# Autodesk Inventor assembly: 1054.000(2)
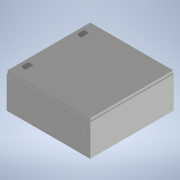
[picture p0: Inventor's stored thumbnail of the model, 180x180]
Saved by Autodesk Inventor 2021 (Build 250183000, 183)
## iProperties
Category: PARTsolutions
Company: RITTAL
Created: 2025-08-26
Part Number: 1054.000(2)
Catalog Web Link: www.cadenas.de
Description: AX Compact enclosure-sheet steel
Vendor: RITTAL
Document SubType Name: Assembly
Designer: psAdmin
Manufacturer: RITTAL
Mass: 3196.97 g
Surface Area: 36267.6 cm^2
Volume: 3196.97 cm^3
Density: 1 g/cm^3
Title: 1054.000(2)
Author: Cadenas PARTsolutions
Comments: sheet steel
PSOL_IDENT_0: {$CADENAS_DATA/23d-libs/rittal/schaltschranksys/kompakt_schaltschr/ae_2_0_asmtab.prj},203 {VTYP=3D},
PSOL_IDENT_1: {STYP=ASSTAB},{NB=1054.000(2)},{LINA=1054.000(2)},{NN=AX Compact enclosure},{DATE=28.04.2025 21:11:2
PSOL_IDENT_2: 3},{GEOMDATE=11.04.2025 11:21:44},{VERSION=},{LINEID=340},{WBVAR=DETAIL},{WBNUMERIC=DETAIL}  {NB=105
PSOL_IDENT_3: 4.000(2)},{LINA=1054.000(2)},{KT=DUMMY},{BEST=1054.000},{BEM=2},{DETAIL=2},{INFOWWW=Website},{BEZ1=A
PSOL_IDENT_4: X Kompakt-Schaltschrank},{BEZ2=Stahlblech},{BEZ3=eintürig},{INFO=Überarbeitete Version 11/2024},{B=6
PSOL_IDENT_5: 00},{H=600},{T=250},{F=550},{G=575},{B1=600},{H1=600},{T1=250},{F1=550},{G1=575},{S=2.5},{ST=MIN},{G
PSOL_IDENT_6: EW=23,4},{VERS=34},{CNSECLASS51=27-18-01-02},{CNSECLASS70=27-18-01-01},{CNSECLASS80=27-18-01-01},{CN
PSOL_IDENT_7: SETIM40=EC000261},{PPATH=assemblies_ae_2_0/ae_2_0_asmtpl.prj},{INFOPAGE=ax_s30},{INFOPATH=http://www
PSOL_IDENT_8: .rittal.com/de-de/part/1054000},{BESTE1=1054},{BESTE2=000},{DETAIL1= 2, 'niedrig', 'detail_2.png', 1
PSOL_IDENT_9: , 'hoch', 'detail_1.png', 11  , 'hochsperr', 'detail_11.png'},{CNSETIM80=EC000261},{CNSETIM90=EC0002
PSOL_IDENT_10: 61},{CNSECLASS60=27-18-01-01},{UNSPSC=31-26-15-02}
NB: 1054.000(2)
NN: AX Compact enclosure
NT: sheet steel
NBSYN: $BEST.($DETAIL.)
LINA: 1054.000(2)
CATALOG: Rittal
BEST: 1054.000
DETAIL: low
INFOWWW: webseite
BEZ1: AX Compact enclosure
BEZ2: sheet steel
BEZ3: single door
INFO: Revised version 11/2024
B: 600
H: 600
T: 250
F: 550
G: 575
GEW: 23,4
CNSECLASS70: 27-18-01-01
CNSECLASS80: 27-18-01-01
CNSETIM80: EC000261
CNSETIM90: EC000261
CNSECLASS60: 27-18-01-01
UNSPSC: 31-26-15-02
SUPPLIER: RITTAL
ARTICLENO: 1054.000(2)
BOMINFO: 1054.000(2)
CREATOR: CADENAS GmbH
## Documents named in this file (9)
- e:\temp\worker_COMMON_247\temp\tmp_5808_86_FYTeN\format_0\1054_000(2).iam
- e:\temp\worker_COMMON_247\temp\tmp_5808_86_FYTeN\format_0\1054_000(2)_P1.ipt
- e:\temp\worker_COMMON_247\temp\tmp_5808_86_FYTeN\format_0\1XXX_01_04(B,2)_P7.ipt
- e:\temp\worker_COMMON_247\temp\tmp_5808_86_FYTeN\format_0\1XXX_01_04(T,2)_P7.ipt
- e:\temp\worker_COMMON_247\temp\tmp_5808_86_FYTeN\format_0\166X_01_01(2)_P2.ipt
- e:\temp\worker_COMMON_247\temp\tmp_5808_86_FYTeN\format_0\1XXX_01_05(2)_P8.ipt
- e:\temp\worker_COMMON_247\temp\tmp_5808_86_FYTeN\format_0\1XX7_04_00_7(2)_P5.ipt
- e:\temp\worker_COMMON_247\temp\tmp_5808_86_FYTeN\format_0\166X_02_00_P6_(2).ipt
- e:\temp\worker_COMMON_247\temp\tmp_5808_86_FYTeN\format_0\0000-00168553(2).ipt
## Components (9 placed, 8 different names)
1. 1054_000(2)_P1:1 — SCRO_XY@1 <-> SC_XY@2, SCRO_Z@1 <-> SC_Z@2, SCRO_YZ@1 <-> SC_YZ@2, SCRU_XY@1 <-> SC_XY@3, SCRU_Z@1 <-> SC_Z@3, SCRU_YZ@1 <-> SC_YZ@3, FP1_XY@1 <-> FP_XY@7, FP1_Z@1 <-> FP_Z@7, FP1_YZ@1 <-> FP_YZ@7, MP_XY@1 <-> MP_XY@8, MP_Z@1 <-> MP_Z@8, MP_YZ@1 <-> MP_YZ@8, to_Plug_XY@1 <-> P1_XY@9, to_Plug_Z@1 <-> P1_Z@9, to_Plug_YZ@1 <-> P1_YZ@9
2. 1XXX_01_04(B,2)_P7:1 — SCRO_XY@1 <-> SC_XY@2, SCRO_Z@1 <-> SC_Z@2, SCRO_YZ@1 <-> SC_YZ@2
3. 1XXX_01_04(T,2)_P7:1 — SCRU_XY@1 <-> SC_XY@3, SCRU_Z@1 <-> SC_Z@3, SCRU_YZ@1 <-> SC_YZ@3, TUER2_XY@3 <-> ET_XY@4, TUER2_Z@3 <-> ET_Z@4
4. 166X_01_01(2)_P2:1 — TUER2_XY@3 <-> ET_XY@4, TUER2_Z@3 <-> ET_Z@4, VV1_XY@4 <-> VV_XY@5, VV1_Z@4 <-> VV_Z@5, VV1_YZ@4 <-> VV_YZ@5, VV2_XY@4 <-> VV_XY@6, VV2_Z@4 <-> VV_Z@6, VV2_YZ@4 <-> VV_YZ@6
5. 1XXX_01_05(2)_P8:1 — VV1_XY@4 <-> VV_XY@5, VV1_Z@4 <-> VV_Z@5, VV1_YZ@4 <-> VV_YZ@5
6. 1XXX_01_05(2)_P8:2 — VV2_XY@4 <-> VV_XY@6, VV2_Z@4 <-> VV_Z@6, VV2_YZ@4 <-> VV_YZ@6
7. 1XX7_04_00_7(2)_P5:1 — FP1_XY@1 <-> FP_XY@7, FP1_Z@1 <-> FP_Z@7, FP1_YZ@1 <-> FP_YZ@7
8. 166X_02_00_P6_(2):1 — MP_XY@1 <-> MP_XY@8, MP_Z@1 <-> MP_Z@8, MP_YZ@1 <-> MP_YZ@8
9. 0000-00168553(2):1 — to_Plug_XY@1 <-> P1_XY@9, to_Plug_Z@1 <-> P1_Z@9, to_Plug_YZ@1 <-> P1_YZ@9
## Relationships (23: Mate 15, Angle 7, Flush 1)
- SCRO_XY@1 <-> SC_XY@2 [Mate]: 1054_000(2)_P1:1 ↔ 1XXX_01_04(B,2)_P7:1
- SCRO_Z@1 <-> SC_Z@2 [Mate]: 1054_000(2)_P1:1 ↔ 1XXX_01_04(B,2)_P7:1
- SCRO_YZ@1 <-> SC_YZ@2 [Angle] (0 deg): 1054_000(2)_P1:1 ↔ 1XXX_01_04(B,2)_P7:1
- SCRU_XY@1 <-> SC_XY@3 [Mate]: 1054_000(2)_P1:1 ↔ 1XXX_01_04(T,2)_P7:1
- SCRU_Z@1 <-> SC_Z@3 [Mate]: 1054_000(2)_P1:1 ↔ 1XXX_01_04(T,2)_P7:1
- SCRU_YZ@1 <-> SC_YZ@3 [Angle] (0 deg): 1054_000(2)_P1:1 ↔ 1XXX_01_04(T,2)_P7:1
- TUER2_XY@3 <-> ET_XY@4 [Mate]: 1XXX_01_04(T,2)_P7:1 ↔ 166X_01_01(2)_P2:1
- TUER2_Z@3 <-> ET_Z@4 [Mate]: 1XXX_01_04(T,2)_P7:1 ↔ 166X_01_01(2)_P2:1
- VV1_XY@4 <-> VV_XY@5 [Mate]: 166X_01_01(2)_P2:1 ↔ 1XXX_01_05(2)_P8:1
- VV1_Z@4 <-> VV_Z@5 [Mate]: 166X_01_01(2)_P2:1 ↔ 1XXX_01_05(2)_P8:1
- VV1_YZ@4 <-> VV_YZ@5 [Angle] (0 deg): 166X_01_01(2)_P2:1 ↔ 1XXX_01_05(2)_P8:1
- VV2_XY@4 <-> VV_XY@6 [Mate]: 166X_01_01(2)_P2:1 ↔ 1XXX_01_05(2)_P8:2
- VV2_Z@4 <-> VV_Z@6 [Mate]: 166X_01_01(2)_P2:1 ↔ 1XXX_01_05(2)_P8:2
- VV2_YZ@4 <-> VV_YZ@6 [Angle] (0 deg): 166X_01_01(2)_P2:1 ↔ 1XXX_01_05(2)_P8:2
- FP1_XY@1 <-> FP_XY@7 [Mate]: 1054_000(2)_P1:1 ↔ 1XX7_04_00_7(2)_P5:1
- FP1_Z@1 <-> FP_Z@7 [Mate]: 1054_000(2)_P1:1 ↔ 1XX7_04_00_7(2)_P5:1
- FP1_YZ@1 <-> FP_YZ@7 [Angle] (0 deg): 1054_000(2)_P1:1 ↔ 1XX7_04_00_7(2)_P5:1
- MP_XY@1 <-> MP_XY@8 [Mate]: 1054_000(2)_P1:1 ↔ 166X_02_00_P6_(2):1
- MP_Z@1 <-> MP_Z@8 [Mate]: 1054_000(2)_P1:1 ↔ 166X_02_00_P6_(2):1
- MP_YZ@1 <-> MP_YZ@8 [Angle] (0 deg): 1054_000(2)_P1:1 ↔ 166X_02_00_P6_(2):1
- to_Plug_XY@1 <-> P1_XY@9 [Flush]: 1054_000(2)_P1:1 ↔ 0000-00168553(2):1
- to_Plug_Z@1 <-> P1_Z@9 [Mate]: 1054_000(2)_P1:1 ↔ 0000-00168553(2):1
- to_Plug_YZ@1 <-> P1_YZ@9 [Angle] (0 deg): 1054_000(2)_P1:1 ↔ 0000-00168553(2):1
